# Autodesk Inventor assembly: RPI and PiTFT
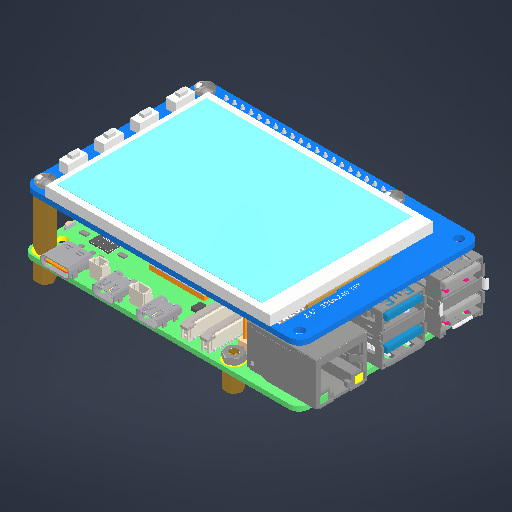
[picture p0: Inventor's stored thumbnail of the model, 512x512]
Saved by Autodesk Inventor 2026 (Build 300175000, 175)
## iProperties
Created: 2025-06-05
Part Number: RPI and PiTFT
Document SubType Name: Assembly
Designer: ckyiu
Author: ckyiu
## Documents named in this file (7)
- F:\Chessboard-Design\Design\Core\PCBs\RPI and PiTFT.iam
- F:\Chessboard-Design\Design\Core\PCBs\Parts\Raspberry Pi 5.iam
- F:\Chessboard-Design\Design\Core\PCBs\Parts\PiTFT 2.8in capacitive.ipt
- F:\Chessboard-Design\Design\Hardware\M2.5\Standoffs\M-F\(6mm) 98952A103_Aluminum Male-Female Threaded Hex Standoff.ipt
- F:\Chessboard-Design\Design\Hardware\M2.5\Standoffs\F-F\(16mm) 95947A011_Aluminum Female Threaded Hex Standoff.ipt
- F:\Chessboard-Design\Design\Hardware\M2.5\Nuts\(2mm) 91828A113_18-8 Stainless Steel Hex Nut.ipt
- F:\Chessboard-Design\Design\Hardware\M2.5\Screws\(6mm) 92000A104_Passivated 18-8 Stainless Steel Pan Head Phillips Screws.ipt
## Components (13 placed, 6 different names)
1. Raspberry Pi 5:1 [sub-assembly] — Flush:1, Mate:1, Flush:2, Insert:1, Insert:2, Insert:4, Insert:5, Insert:7, Insert:8, Insert:9, Insert:10
2. PiTFT 2.8in capacitive:1 — Flush:1, Mate:1, Flush:2, Insert:3, Insert:6, Insert:11
3. (6mm) 98952A103_Aluminum Male-Female Threaded Hex Standoff:1 — Insert:1
4. (6mm) 98952A103_Aluminum Male-Female Threaded Hex Standoff:2 — Insert:9
5. (6mm) 98952A103_Aluminum Male-Female Threaded Hex Standoff:3 — Insert:4
6. (6mm) 98952A103_Aluminum Male-Female Threaded Hex Standoff:4 — Insert:7
7. (2mm) 91828A113_18-8 Stainless Steel Hex Nut:1 — Insert:8
8. (16mm) 95947A011_Aluminum Female Threaded Hex Standoff:1 — Insert:10
9. (16mm) 95947A011_Aluminum Female Threaded Hex Standoff:2 — Insert:2
10. (16mm) 95947A011_Aluminum Female Threaded Hex Standoff:3 — Insert:5
11. (6mm) 92000A104_Passivated 18-8 Stainless Steel Pan Head Phillips Screws:1 — Insert:11
12. (6mm) 92000A104_Passivated 18-8 Stainless Steel Pan Head Phillips Screws:2 — Insert:3
13. (6mm) 92000A104_Passivated 18-8 Stainless Steel Pan Head Phillips Screws:3 — Insert:6
## Relationships (14: Insert 11, Flush 2, Mate 1)
- Flush:1: Raspberry Pi 5:1 ↔ PiTFT 2.8in capacitive:1
- Mate:1: Raspberry Pi 5:1 ↔ PiTFT 2.8in capacitive:1
- Flush:2: Raspberry Pi 5:1 ↔ PiTFT 2.8in capacitive:1
- Insert:1: Raspberry Pi 5:1 ↔ (6mm) 98952A103_Aluminum Male-Female Threaded Hex Standoff:1
- Insert:2: Raspberry Pi 5:1 ↔ (16mm) 95947A011_Aluminum Female Threaded Hex Standoff:2
- Insert:3: PiTFT 2.8in capacitive:1 ↔ (6mm) 92000A104_Passivated 18-8 Stainless Steel Pan Head Phillips Screws:2
- Insert:4: Raspberry Pi 5:1 ↔ (6mm) 98952A103_Aluminum Male-Female Threaded Hex Standoff:3
- Insert:5: Raspberry Pi 5:1 ↔ (16mm) 95947A011_Aluminum Female Threaded Hex Standoff:3
- Insert:6: PiTFT 2.8in capacitive:1 ↔ (6mm) 92000A104_Passivated 18-8 Stainless Steel Pan Head Phillips Screws:3
- Insert:7: Raspberry Pi 5:1 ↔ (6mm) 98952A103_Aluminum Male-Female Threaded Hex Standoff:4
- Insert:8: Raspberry Pi 5:1 ↔ (2mm) 91828A113_18-8 Stainless Steel Hex Nut:1
- Insert:9: Raspberry Pi 5:1 ↔ (6mm) 98952A103_Aluminum Male-Female Threaded Hex Standoff:2
- Insert:10: Raspberry Pi 5:1 ↔ (16mm) 95947A011_Aluminum Female Threaded Hex Standoff:1
- Insert:11: PiTFT 2.8in capacitive:1 ↔ (6mm) 92000A104_Passivated 18-8 Stainless Steel Pan Head Phillips Screws:1
